# Autodesk Inventor assembly: Eje_Engrane-llanta
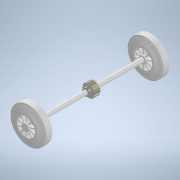
[picture p0: Inventor's stored thumbnail of the model, 180x180]
Saved by Autodesk Inventor 2021 (Build 250183000, 183)
## iProperties
Created: 2021-02-07
Part Number: Eje_Engrane-llanta
Document SubType Name: Assembly
Designer: rotje
Author: rotje
## Documents named in this file (4)
- C:\Users\rotje\Documents\Inventor\MSF\Eje_Engrane-llanta.iam
- C:\Users\rotje\Documents\Inventor\MSF\Eje_Engranes_llanta.ipt
- C:\Users\rotje\Documents\Inventor\MSF\Engranaje recto_20_Dientes.ipt
- C:\Users\rotje\Documents\Inventor\MSF\Llanta_125-15.ipt
## Components (4 placed, 3 different names)
1. Eje_Engranes_llanta:1 — Insertar:1, Insertar:2, Insertar:3
2. Engranaje recto1:1 — Insertar:1
3. Llanta_125-15:1 — Insertar:3
4. Llanta_125-15:2 — Insertar:2
## Relationships (3: Insert 3)
- Insertar:1: Eje_Engranes_llanta:1 ↔ Engranaje recto1:1
- Insertar:2: Eje_Engranes_llanta:1 ↔ Llanta_125-15:2
- Insertar:3: Eje_Engranes_llanta:1 ↔ Llanta_125-15:1
